# Autodesk Inventor assembly: SwitchMatrix_PCB
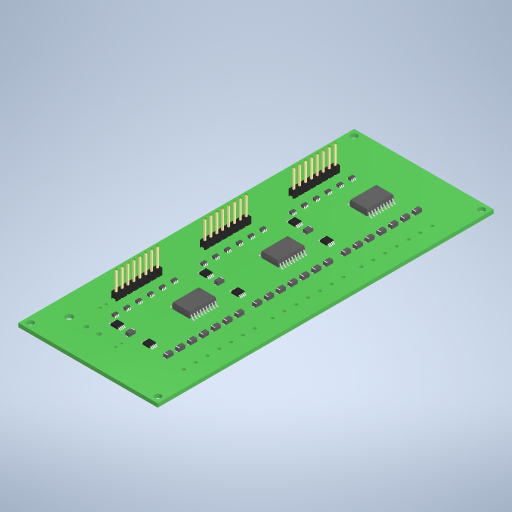
[picture p0: Inventor's stored thumbnail of the model, 512x512]
Saved by Autodesk Inventor 2023.1 (Build 271208000, 208)
## iProperties
Created: 2022-07-14
Part Number: SwitchMatrix_PCB
Document SubType Name: Assembly
Designer: jirlowm
Author: jirlowm
## iProperties of the stored document TBD62781AFWG,EL.iam
Created: 2022-07-14
Part Number: TBD62781AFWG,EL
Document SubType Name: Assembly
Designer: jirlowm
Author: jirlowm
## iProperties of the stored document COMPOUND_1.ipt
Created: 2022-07-14
Part Number: COMPOUND
Material: Generic
Document SubType Name: Modeling
Designer: jirlowm
Density: 1 g/cm^3
Appearance: Default
Author: jirlowm
## iProperties of the stored document switch_matrix_dist_board.iam
Company: Kicad
Created: 2022-07-14
Part Number: switch_matrix_dist_board 1
Description: KiCad electronic assembly
Document SubType Name: Assembly
Designer: jirlowm
Authority: Unknown
Sending System: KiCad to STEP converter
Preprocessor: Open CASCADE STEP processor 7.6
Title: switch_matrix_dist_board.step
Author: Pcbnew
## iProperties of the stored document TMUX1248DCKR.iam
Created: 2022-07-14
Part Number: TMUX1248DCKR
Document SubType Name: Assembly
Designer: jirlowm
Author: jirlowm
## iProperties of the stored document COMPOUND_2.ipt
Created: 2022-07-14
Part Number: COMPOUND
Material: Generic
Document SubType Name: Modeling
Designer: jirlowm
Density: 1 g/cm^3
Appearance: Default
Author: jirlowm
## iProperties of the stored document COMPOUND.ipt
Created: 2022-07-14
Part Number: COMPOUND
Material: Generic
Document SubType Name: Modeling
Designer: jirlowm
Density: 1 g/cm^3
Appearance: Default
Author: jirlowm
## iProperties of the stored document SM4003PL-TP.iam
Created: 2022-07-14
Part Number: SM4003PL-TP
Document SubType Name: Assembly
Designer: jirlowm
Author: jirlowm
## iProperties of the stored document switch_matrix_dist_board PCB.ipt
Created: 2022-07-14
Part Number: switch_matrix_dist_board PCB
Material: Generic
Document SubType Name: Modeling
Designer: jirlowm
Density: 1 g/cm^3
Appearance: Default
Author: jirlowm
## iProperties of the stored document TMUX6219DGKRQ1.iam
Created: 2022-07-14
Part Number: TMUX6219DGKRQ1
Document SubType Name: Assembly
Designer: jirlowm
Author: jirlowm
## iProperties of the stored document COMPOUND_3.ipt
Created: 2022-07-14
Part Number: COMPOUND
Material: Generic
Document SubType Name: Modeling
Designer: jirlowm
Density: 1 g/cm^3
Appearance: Default
Author: jirlowm
## Documents named in this file (14)
- C:\Users\jirlowm\Documents\Inventor\SwitchMatrix\SwitchMatrix_PCB.iam
- **C:\Users\jirlowm\Documents\Inventor\SwitchMatrix\SwitchMatrix_PCB.iam*LocalDocs*xAaaaa4caAaaaaaaaAaaaa31bCg*switch_matrix_dist_board.iam
- C:\Users\jirlowm\Documents\Inventor\SwitchMatrix\SwitchMatrix_PCB\AIP\Cable and Harness\SwitchMatrix_PCB.Harness1.iam
- C:\Users\jirlowm\Documents\Inventor\SwitchMatrix\Pin Headers\1x8 Male Pin Header.ipt
- **C:\Users\jirlowm\Documents\Inventor\SwitchMatrix\SwitchMatrix_PCB.iam*LocalDocs*xAaaaq0daAaaaaaaaAaaaqtr0Ng*TBD62781AFWG,EL.iam
- **C:\Users\jirlowm\Documents\Inventor\SwitchMatrix\SwitchMatrix_PCB.iam*LocalDocs*xAaaaqnaaAaaaaaaaAaaaqfke2d*COMPOUND_3.ipt
- **C:\Users\jirlowm\Documents\Inventor\SwitchMatrix\SwitchMatrix_PCB.iam*LocalDocs*xAaaaamdaAaaaaaaaAaaaacedKb*COMPOUND_1.ipt
- **C:\Users\jirlowm\Documents\Inventor\SwitchMatrix\SwitchMatrix_PCB.iam*LocalDocs*xAaaaqidaAaaaaaaaAaaaafr01c*SM4003PL-TP.iam
- **C:\Users\jirlowm\Documents\Inventor\SwitchMatrix\SwitchMatrix_PCB.iam*LocalDocs*xAaaaasbaAaaaaaaaAaaaa1mt2e*TMUX1248DCKR.iam
- **C:\Users\jirlowm\Documents\Inventor\SwitchMatrix\SwitchMatrix_PCB.iam*LocalDocs*xAaaaqkbaAaaaaaaaAaaaqu3y3b*TMUX6219DGKRQ1.iam
- **C:\Users\jirlowm\Documents\Inventor\SwitchMatrix\SwitchMatrix_PCB.iam*LocalDocs*xAaaaqcaaAaaaaaaaAaaaqdzf0a*switch_matrix_dist_board PCB.ipt
- **C:\Users\jirlowm\Documents\Inventor\SwitchMatrix\SwitchMatrix_PCB.iam*LocalDocs*xAaaaq5baAaaaaaaaAaaaaookDh*COMPOUND_2.ipt
- **C:\Users\jirlowm\Documents\Inventor\SwitchMatrix\SwitchMatrix_PCB.iam*LocalDocs*xAaaaq2aaAaaaaaaaAaaaqjo0Ab*COMPOUND.ipt
- C:\Users\jirlowm\Documents\CAD Models\switch_matrix_dist_board.step
## Components (5 placed, 3 different names)
1. switch_matrix_dist_board:1 [sub-assembly] — Mate:20, Mate:21, Mate:22
2. Harness1 [sub-assembly]
3. 1x8 Male Pin Header:1 — Mate:20
4. 1x8 Male Pin Header:2 — Mate:21
5. 1x8 Male Pin Header:3 — Mate:22
## Relationships (3: Mate 3)
- Mate:20: switch_matrix_dist_board:1 ↔ 1x8 Male Pin Header:1
- Mate:21: switch_matrix_dist_board:1 ↔ 1x8 Male Pin Header:2
- Mate:22: switch_matrix_dist_board:1 ↔ 1x8 Male Pin Header:3
